# Autodesk Inventor assembly: SensorAssembly
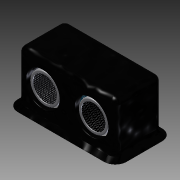
[picture p0: Inventor's stored thumbnail of the model, 180x180]
Saved by Autodesk Inventor 2014 SP2 (Build 180246200, 246)
## iProperties
Created: 2020-01-02
Part Number: SensorAssembly
Document SubType Name: Assembly
Designer: GauchoHP
Author: GauchoHP
## Documents named in this file (3)
- C:\Users\GauchoHP\Desktop\old_desktop\tosaerba\LAWNMOWER-ROBOT-from-Hoverboard-\LawnmowerMechanicalProject\3D PROJECT - INVENTOR 2014\sensors\SensorAssembly.iam
- C:\Users\GauchoHP\Desktop\old_desktop\tosaerba\LAWNMOWER-ROBOT-from-Hoverboard-\LawnmowerMechanicalProject\3D PROJECT - INVENTOR 2014\sensors\support\base.ipt
- C:\Users\GauchoHP\Desktop\old_desktop\tosaerba\LAWNMOWER-ROBOT-from-Hoverboard-\LawnmowerMechanicalProject\3D PROJECT - INVENTOR 2014\sensors\sensor\HC-SR04.iam
## Components (2 placed, 2 different names)
1. base:1 — Mate:1, Mate:2, Flush:1
2. HC-SR04:2 [sub-assembly] — Mate:1, Mate:2, Flush:1
## Relationships (3: Mate 2, Flush 1)
- Mate:1 (10 mm): base:1 ↔ HC-SR04:2
- Mate:2 (-1 mm): base:1 ↔ HC-SR04:2
- Flush:1 (4 mm): base:1 ↔ HC-SR04:2
